# Autodesk Inventor assembly: link3
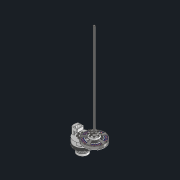
[picture p0: Inventor's stored thumbnail of the model, 180x180]
Saved by Autodesk Inventor 2022 (Build 260153000, 153)
## iProperties
Created: 2021-10-13
Part Number: link3
Document SubType Name: Assembly
Designer: Yuta Kage
Author: Yuta Kage
## Documents named in this file (2)
- C:\Users\yuta0\Documents\GitHub\catchrobo_hardware\mesh\scara\link3.iam
- C:\Users\yuta0\Documents\GitHub\catchrobo_hardware\assy-scara\s-assy-linear_joint.iam
## Components (1 placed, 1 different names)
1. s-assy-linear_joint:3 [sub-assembly] — フラッシュ:1, メイト:1, フラッシュ:2
## Relationships (3: Flush 2, Mate 1)
- フラッシュ:1 [Flush]: s-assy-linear_joint:3
- メイト:1 [Mate]: s-assy-linear_joint:3
- フラッシュ:2 [Flush] (-15.05 mm): s-assy-linear_joint:3
